# Autodesk Inventor assembly: 分析報告用
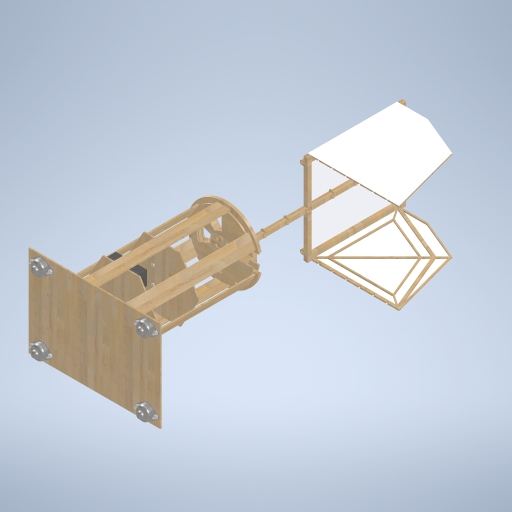
[picture p0: Inventor's stored thumbnail of the model, 512x512]
Saved by Autodesk Inventor 2024 (Build 280153000, 153)
## iProperties
Created: 2024-04-09
Part Number: 分析報告用
Document SubType Name: Assembly
Designer: USER
Author: USER
## Documents named in this file (28)
- C:\文件\機械工程實務\3D_CAD_Drawing\[Midterm]Design\分析報告用.iam
- C:\文件\機械工程實務\3D_CAD_Drawing\[Midterm]Design\cow_wheel.ipt
- C:\文件\機械工程實務\3D_CAD_Drawing\[Midterm]Design\back_down_hold.ipt
- C:\文件\機械工程實務\3D_CAD_Drawing\[Midterm]Design\back_cir_hold.ipt
- C:\文件\機械工程實務\3D_CAD_Drawing\[Midterm]Design\middle_space.ipt
- C:\文件\機械工程實務\3D_CAD_Drawing\[Midterm]Design\rolling_plate.ipt
- C:\文件\機械工程實務\3D_CAD_Drawing\[Midterm]Design\rolling_plate_top.ipt
- C:\文件\機械工程實務\3D_CAD_Drawing\[Midterm]Design\rolling_plate_small.ipt
- C:\文件\機械工程實務\3D_CAD_Drawing\[Midterm]Design\左右.ipt
- C:\文件\機械工程實務\3D_CAD_Drawing\[Midterm]Design\左右2.ipt
- C:\文件\機械工程實務\3D_CAD_Drawing\[Midterm]Design\馬達.ipt
- C:\文件\機械工程實務\3D_CAD_Drawing\[Midterm]Design\軸.ipt
- C:\文件\機械工程實務\3D_CAD_Drawing\[Midterm]Design\螺絲.ipt
- C:\文件\機械工程實務\3D_CAD_Drawing\[Midterm]Design\Base_final.ipt
- C:\文件\機械工程實務\3D_CAD_Drawing\[Midterm]Design\sail(Midterm).iam
- C:\文件\機械工程實務\3D_CAD_Drawing\[Midterm]Design\插銷B.ipt
- C:\文件\機械工程實務\3D_CAD_Drawing\[Midterm]Design\插銷A.ipt
- C:\文件\機械工程實務\3D_CAD_Drawing\[Midterm]Design\機電設備\18650電池盒\18650電池盒.ipt
- C:\文件\機械工程實務\3D_CAD_Drawing\[Midterm]Design\機電設備\馬達驅動模組\馬達驅動模組.ipt
- C:\文件\機械工程實務\3D_CAD_Drawing\[Midterm]Design\機電設備\銅柱\銅柱.ipt
- C:\文件\機械工程實務\3D_CAD_Drawing\[Midterm]Design\機電設備\Arduino板\Arduino板.iam
- C:\文件\機械工程實務\3D_CAD_Drawing\[Midterm]Design\機電設備\麵包板\麵包板.ipt
- C:\文件\機械工程實務\3D_CAD_Drawing\[Midterm]Design\機電設備\9V方型電池盒\9V方型電池盒.ipt
- C:\文件\機械工程實務\3D_CAD_Drawing\[Midterm]Design\m4螺栓.ipt
- C:\文件\機械工程實務\3D_CAD_Drawing\[Midterm]Design\middle_space2.ipt
- C:\文件\機械工程實務\3D_CAD_Drawing\[Midterm]Design\機電設備\M3螺帽\M3螺帽.ipt
- C:\文件\機械工程實務\3D_CAD_Drawing\[Midterm]Design\機電設備\M3螺栓\M3螺栓.ipt
- C:\文件\機械工程實務\3D_CAD_Drawing\[Midterm]Design\M4螺帽.ipt
## Components (70 placed, 27 different names)
1. cow_wheel:1 — 貼合:82, 貼合:83, 貼合:84, 插入:25, 插入:26
2. cow_wheel:2 — 貼合:86, 貼合:156, 貼合:157, 插入:23, 插入:24
3. cow_wheel:3 — 貼合:80, 貼合:81, 貼合:85, 插入:12, 插入:14
4. cow_wheel:4 — 貼合:75, 貼合:76, 貼合:77, 貼合:78, 貼合:79, 插入:27, 插入:28
5. back_down_hold:1 — 貼合:99, 貼合:100, 貼合:101, 貼合:102, 貼合:147
6. back_down_hold:2 — 貼合:34, 齊平:14, 相切:1, 齊平:28, 貼合:92, 貼合:93, 貼合:94
7. back_down_hold:3 — 齊平:5, 齊平:13, 貼合:90, 貼合:91, 貼合:149
8. back_down_hold:4 — 貼合:87, 貼合:97, 貼合:98
9. back_down_hold:5 — 齊平:6, 貼合:48, 貼合:88, 貼合:89, 貼合:105, 貼合:148, 齊平:44, 貼合:150, 貼合:151
10. back_down_hold:6 — 齊平:5, 齊平:6, 貼合:32, 貼合:33, 貼合:95, 貼合:96, 貼合:146, 角度:3
11. back_cir_hold:1 — 貼合:32, 貼合:33, 貼合:34, 貼合:104, 角度:1, 貼合:109
12. middle_space:1 — 齊平:13, 貼合:48, 齊平:14, 齊平:28, 貼合:145
13. rolling_plate:2 — 貼合:56, 貼合:57, 齊平:24, 貼合:104, 貼合:108, 貼合:109, 齊平:31, 貼合:135, 貼合:136, 貼合:139, 貼合:140, 貼合:141
14. rolling_plate_top:1 — 相切:1, 貼合:58, 貼合:59, 貼合:60, 貼合:61, 貼合:62, 貼合:63, 角度:1, 貼合:108, 貼合:113, 貼合:114, 貼合:115, 貼合:116, 貼合:117, 齊平:30, 貼合:118, 貼合:119, 貼合:120, 貼合:121, 貼合:122, 貼合:123, 貼合:124, 貼合:125, 貼合:126, 貼合:128, 貼合:129, 貼合:131, 貼合:132, 貼合:133, 貼合:137
15. rolling_plate_small:1 — 貼合:52, 齊平:16, 齊平:19, 貼合:56, 齊平:24
16. rolling_plate_small:2 — 貼合:52, 齊平:16, 齊平:19, 貼合:57, 貼合:107, 齊平:29
17. rolling_plate_small:4 — 貼合:107, 齊平:29, 貼合:116, 貼合:117, 齊平:30
18. 左右:1 — 貼合:58, 貼合:59, 貼合:60, 貼合:66, 貼合:67, 齊平:26, 貼合:68, 齊平:27
19. 左右2:1 — 貼合:61, 貼合:62, 貼合:63, 角度:2
20. 馬達:1 — 貼合:64, 貼合:65, 貼合:69, 貼合:70, 貼合:71
21. 軸:1 — 貼合:64, 貼合:65, 貼合:110, 貼合:111, 貼合:112
22. 螺絲:1 — 齊平:25, 貼合:66, 貼合:67, 齊平:26, 貼合:69, 貼合:70
23. 螺絲:2 — 齊平:25, 貼合:68, 齊平:27, 貼合:71
24. Base_final:1 — 貼合:75, 貼合:76, 貼合:77, 貼合:78, 貼合:79, 貼合:80, 貼合:81, 貼合:82, 貼合:83, 貼合:84, 貼合:85, 貼合:86, 貼合:87, 貼合:88, 貼合:89, 貼合:90, 貼合:91, 貼合:92, 貼合:93, 貼合:94, 貼合:95, 貼合:96, 貼合:97, 貼合:98, 貼合:99, 貼合:100, 貼合:101, 貼合:102, 貼合:105, 貼合:142, 貼合:143, 貼合:144, 齊平:40, 齊平:41, 齊平:42, 齊平:43, 插入:15, 插入:16, 插入:17, 插入:18, 插入:19, 插入:20, 插入:21, 插入:22, 貼合:156, 貼合:157
25. sail(Midterm):1 [sub-assembly] — 貼合:110, 貼合:111, 貼合:112, 角度:2
26. 插銷A:1 — 齊平:32, 貼合:127, 齊平:33, 貼合:128
27. 插銷B:2 — 貼合:123, 貼合:124, 貼合:125
28. 插銷A:2 — 貼合:138, 齊平:38, 齊平:39, 貼合:141
29. 插銷B:3 — 貼合:121, 齊平:31, 貼合:122
30. 插銷A:3 — 貼合:130, 齊平:34, 齊平:35, 貼合:131
31. 插銷B:4 — 貼合:118, 貼合:119, 貼合:120
32. 插銷A:5 — 貼合:126, 齊平:32, 貼合:127, 齊平:33, 貼合:129
33. 插銷B:6 — 貼合:113, 貼合:114, 貼合:115
34. 插銷A:6 — 貼合:134, 齊平:36, 齊平:37, 貼合:135, 貼合:136
35. 插銷A:7 — 貼合:130, 齊平:34, 齊平:35, 貼合:132, 貼合:133
36. 插銷A:8 — 貼合:138, 齊平:38, 齊平:39, 貼合:139, 貼合:140
37. 插銷A:9 — 貼合:134, 齊平:36, 齊平:37, 貼合:137
38. 18650電池盒:1 — 貼合:143, 貼合:146, 貼合:147
39. 馬達驅動模組:1 — 插入:6, 角度:3, 貼合:152, 插入:7, 貼合:154, 貼合:155
40. 銅柱:1 — 插入:2
41. Arduino板:1 [sub-assembly] — 貼合:142, 齊平:40, 齊平:41
42. 麵包板:1 — 貼合:144, 齊平:42, 齊平:43
43. 9V方型電池盒:1 — 貼合:145, 貼合:148, 貼合:149
44. middle_space2:1 — 齊平:44, 貼合:150, 貼合:151, 插入:2, 插入:3, 插入:4, 插入:5, 插入:9, 插入:10, 插入:11
45. 銅柱:2 — 插入:4, 插入:6
46. 銅柱:3 — 插入:5
47. 銅柱:4 — 插入:3, 貼合:153
48. M3螺栓:1 — 貼合:152, 貼合:153
49. M4螺帽:2 — 插入:12
50. M3螺栓:2 — 插入:7
51. M3螺栓:3 — 貼合:154
52. M3螺栓:4 — 貼合:155
53. M3螺帽:2 — 插入:9
54. M3螺帽:3 — 插入:10
55. M3螺帽:4 — 插入:11
56. M4螺帽:3 — 插入:14
57. M4螺帽:4 — 插入:23
58. M4螺帽:5 — 插入:24
59. m4螺栓:1 — 插入:15
60. m4螺栓:2 — 插入:16
61. m4螺栓:3 — 插入:19
62. m4螺栓:4 — 插入:20
63. m4螺栓:5 — 插入:17
64. m4螺栓:6 — 插入:18
65. m4螺栓:7 — 插入:22
66. m4螺栓:8 — 插入:21
67. M4螺帽:6 — 插入:25
68. M4螺帽:7 — 插入:26
69. M4螺帽:8 — 插入:27
70. M4螺帽:9 — 插入:28
## Relationships (158: Mate 102, Flush 27, Insert 25, Angle 3, Tangent 1)
- 齊平:5 [Flush]: back_down_hold:3 ↔ back_down_hold:6
- 齊平:6 [Flush]: back_down_hold:5 ↔ back_down_hold:6
- 貼合:32 [Mate]: back_down_hold:6 ↔ back_cir_hold:1
- 貼合:33 [Mate]: back_down_hold:6 ↔ back_cir_hold:1
- 貼合:34 [Mate]: back_down_hold:2 ↔ back_cir_hold:1
- 齊平:13 [Flush]: back_down_hold:3 ↔ middle_space:1
- 貼合:48 [Mate]: back_down_hold:5 ↔ middle_space:1
- 齊平:14 [Flush]: back_down_hold:2 ↔ middle_space:1
- 相切:1 [Tangent]: back_down_hold:2 ↔ rolling_plate_top:1
- 貼合:52 [Mate]: rolling_plate_small:1 ↔ rolling_plate_small:2
- 齊平:16 [Flush]: rolling_plate_small:1 ↔ rolling_plate_small:2
- 齊平:19 [Flush]: rolling_plate_small:1 ↔ rolling_plate_small:2
- 貼合:56 [Mate]: rolling_plate:2 ↔ rolling_plate_small:1
- 貼合:57 [Mate]: rolling_plate:2 ↔ rolling_plate_small:2
- 齊平:24 [Flush]: rolling_plate:2 ↔ rolling_plate_small:1
- 貼合:58 [Mate]: rolling_plate_top:1 ↔ 左右:1
- 貼合:59 [Mate]: rolling_plate_top:1 ↔ 左右:1
- 貼合:60 [Mate]: rolling_plate_top:1 ↔ 左右:1
- 貼合:61 [Mate]: rolling_plate_top:1 ↔ 左右2:1
- 貼合:62 [Mate]: rolling_plate_top:1 ↔ 左右2:1
- 貼合:63 [Mate]: rolling_plate_top:1 ↔ 左右2:1
- 貼合:64 [Mate]: 馬達:1 ↔ 軸:1
- 貼合:65 [Mate]: 馬達:1 ↔ 軸:1
- 齊平:25 [Flush]: 螺絲:1 ↔ 螺絲:2
- 貼合:66 [Mate]: 左右:1 ↔ 螺絲:1
- 貼合:67 [Mate]: 左右:1 ↔ 螺絲:1
- 齊平:26 [Flush]: 左右:1 ↔ 螺絲:1
- 貼合:68 [Mate]: 左右:1 ↔ 螺絲:2
- 齊平:27 [Flush]: 左右:1 ↔ 螺絲:2
- 貼合:69 [Mate]: 馬達:1 ↔ 螺絲:1
- 貼合:70 [Mate]: 馬達:1 ↔ 螺絲:1
- 貼合:71 [Mate]: 馬達:1 ↔ 螺絲:2
- 齊平:28 [Flush]: back_down_hold:2 ↔ middle_space:1
- 貼合:75 [Mate]: cow_wheel:4 ↔ Base_final:1
- 貼合:76 [Mate]: cow_wheel:4 ↔ Base_final:1
- 貼合:77 [Mate]: cow_wheel:4 ↔ Base_final:1
- 貼合:78 [Mate]: cow_wheel:4 ↔ Base_final:1
- 貼合:79 [Mate]: cow_wheel:4 ↔ Base_final:1
- 貼合:80 [Mate]: cow_wheel:3 ↔ Base_final:1
- 貼合:81 [Mate]: cow_wheel:3 ↔ Base_final:1
- 貼合:82 [Mate]: cow_wheel:1 ↔ Base_final:1
- 貼合:83 [Mate]: cow_wheel:1 ↔ Base_final:1
- 貼合:84 [Mate]: cow_wheel:1 ↔ Base_final:1
- 貼合:85 [Mate]: cow_wheel:3 ↔ Base_final:1
- 貼合:86 [Mate]: cow_wheel:2 ↔ Base_final:1
- 貼合:87 [Mate]: back_down_hold:4 ↔ Base_final:1
- 貼合:88 [Mate]: back_down_hold:5 ↔ Base_final:1
- 貼合:89 [Mate]: back_down_hold:5 ↔ Base_final:1
- 貼合:90 [Mate]: back_down_hold:3 ↔ Base_final:1
- 貼合:91 [Mate]: back_down_hold:3 ↔ Base_final:1
- 貼合:92 [Mate]: back_down_hold:2 ↔ Base_final:1
- 貼合:93 [Mate]: back_down_hold:2 ↔ Base_final:1
- 貼合:94 [Mate]: back_down_hold:2 ↔ Base_final:1
- 貼合:95 [Mate]: back_down_hold:6 ↔ Base_final:1
- 貼合:96 [Mate]: back_down_hold:6 ↔ Base_final:1
- 貼合:97 [Mate]: back_down_hold:4 ↔ Base_final:1
- 貼合:98 [Mate]: back_down_hold:4 ↔ Base_final:1
- 貼合:99 [Mate]: back_down_hold:1 ↔ Base_final:1
- 貼合:100 [Mate]: back_down_hold:1 ↔ Base_final:1
- 貼合:101 [Mate]: back_down_hold:1 ↔ Base_final:1
- 貼合:102 [Mate]: back_down_hold:1 ↔ Base_final:1
- 貼合:104 [Mate]: back_cir_hold:1 ↔ rolling_plate:2
- 貼合:105 [Mate]: back_down_hold:5 ↔ Base_final:1
- 角度:1 [Angle] (0 deg): back_cir_hold:1 ↔ rolling_plate_top:1
- 貼合:107 [Mate]: rolling_plate_small:2 ↔ rolling_plate_small:4
- 貼合:108 [Mate]: rolling_plate:2 ↔ rolling_plate_top:1
- 齊平:29 [Flush]: rolling_plate_small:2 ↔ rolling_plate_small:4
- 貼合:109 [Mate] (1.5 mm): back_cir_hold:1 ↔ rolling_plate:2
- 貼合:110 [Mate]: 軸:1 ↔ sail(Midterm):1
- 貼合:111 [Mate]: 軸:1 ↔ sail(Midterm):1
- 貼合:112 [Mate]: 軸:1 ↔ sail(Midterm):1
- 貼合:113 [Mate]: rolling_plate_top:1 ↔ 插銷B:6
- 貼合:114 [Mate]: rolling_plate_top:1 ↔ 插銷B:6
- 貼合:115 [Mate]: rolling_plate_top:1 ↔ 插銷B:6
- 貼合:116 [Mate]: rolling_plate_top:1 ↔ rolling_plate_small:4
- 貼合:117 [Mate]: rolling_plate_top:1 ↔ rolling_plate_small:4
- 齊平:30 [Flush]: rolling_plate_top:1 ↔ rolling_plate_small:4
- 貼合:118 [Mate]: rolling_plate_top:1 ↔ 插銷B:4
- 貼合:119 [Mate]: rolling_plate_top:1 ↔ 插銷B:4
- 貼合:120 [Mate]: rolling_plate_top:1 ↔ 插銷B:4
- 貼合:121 [Mate]: rolling_plate_top:1 ↔ 插銷B:3
- 齊平:31 [Flush]: rolling_plate:2 ↔ 插銷B:3
- 貼合:122 [Mate]: rolling_plate_top:1 ↔ 插銷B:3
- 貼合:123 [Mate]: rolling_plate_top:1 ↔ 插銷B:2
- 貼合:124 [Mate]: rolling_plate_top:1 ↔ 插銷B:2
- 貼合:125 [Mate]: rolling_plate_top:1 ↔ 插銷B:2
- 貼合:126 [Mate]: rolling_plate_top:1 ↔ 插銷A:5
- 齊平:32 [Flush]: 插銷A:1 ↔ 插銷A:5
- 貼合:127 [Mate]: 插銷A:1 ↔ 插銷A:5
- 齊平:33 [Flush]: 插銷A:1 ↔ 插銷A:5
- 貼合:128 [Mate]: rolling_plate_top:1 ↔ 插銷A:1
- 貼合:129 [Mate]: rolling_plate_top:1 ↔ 插銷A:5
- 貼合:130 [Mate]: 插銷A:3 ↔ 插銷A:7
- 齊平:34 [Flush]: 插銷A:3 ↔ 插銷A:7
- 齊平:35 [Flush]: 插銷A:3 ↔ 插銷A:7
- 貼合:131 [Mate]: rolling_plate_top:1 ↔ 插銷A:3
- 貼合:132 [Mate]: rolling_plate_top:1 ↔ 插銷A:7
- 貼合:133 [Mate]: rolling_plate_top:1 ↔ 插銷A:7
- 貼合:134 [Mate]: 插銷A:6 ↔ 插銷A:9
- 齊平:36 [Flush]: 插銷A:6 ↔ 插銷A:9
- 齊平:37 [Flush]: 插銷A:6 ↔ 插銷A:9
- 貼合:135 [Mate]: rolling_plate:2 ↔ 插銷A:6
- 貼合:136 [Mate]: rolling_plate:2 ↔ 插銷A:6
- 貼合:137 [Mate]: rolling_plate_top:1 ↔ 插銷A:9
- 貼合:138 [Mate]: 插銷A:2 ↔ 插銷A:8
- 齊平:38 [Flush]: 插銷A:2 ↔ 插銷A:8
- 齊平:39 [Flush]: 插銷A:2 ↔ 插銷A:8
- 貼合:139 [Mate]: rolling_plate:2 ↔ 插銷A:8
- 貼合:140 [Mate]: rolling_plate:2 ↔ 插銷A:8
- 貼合:141 [Mate]: rolling_plate:2 ↔ 插銷A:2
- 角度:2 [Angle] (0 deg): 左右2:1 ↔ sail(Midterm):1
- 貼合:142 [Mate]: Base_final:1 ↔ Arduino板:1
- 貼合:143 [Mate]: Base_final:1 ↔ 18650電池盒:1
- 貼合:144 [Mate]: Base_final:1 ↔ 麵包板:1
- 貼合:145 [Mate]: middle_space:1 ↔ 9V方型電池盒:1
- 齊平:40 [Flush] (40 mm): Base_final:1 ↔ Arduino板:1
- 齊平:41 [Flush] (30 mm): Base_final:1 ↔ Arduino板:1
- 齊平:42 [Flush] (55 mm): Base_final:1 ↔ 麵包板:1
- 齊平:43 [Flush] (25 mm): Base_final:1 ↔ 麵包板:1
- 貼合:146 [Mate] (30.7 mm): back_down_hold:6 ↔ 18650電池盒:1
- 貼合:147 [Mate] (27.422 mm): back_down_hold:1 ↔ 18650電池盒:1
- 貼合:148 [Mate]: back_down_hold:5 ↔ 9V方型電池盒:1
- 貼合:149 [Mate] (19.072 mm): back_down_hold:3 ↔ 9V方型電池盒:1
- 齊平:44 [Flush]: back_down_hold:5 ↔ middle_space2:1
- 貼合:150 [Mate]: back_down_hold:5 ↔ middle_space2:1
- 貼合:151 [Mate]: back_down_hold:5 ↔ middle_space2:1
- 插入:2 [Insert]: 銅柱:1 ↔ middle_space2:1
- 插入:3 [Insert]: middle_space2:1 ↔ 銅柱:4
- 插入:4 [Insert]: middle_space2:1 ↔ 銅柱:2
- 插入:5 [Insert]: middle_space2:1 ↔ 銅柱:3
- 插入:6 [Insert]: 馬達驅動模組:1 ↔ 銅柱:2
- 角度:3 [Angle] (180 deg): back_down_hold:6 ↔ 馬達驅動模組:1
- 貼合:152 [Mate]: 馬達驅動模組:1 ↔ M3螺栓:1
- 貼合:153 [Mate]: 銅柱:4 ↔ M3螺栓:1
- 插入:7 [Insert]: 馬達驅動模組:1 ↔ M3螺栓:2
- 貼合:154 [Mate]: 馬達驅動模組:1 ↔ M3螺栓:3
- 貼合:155 [Mate]: 馬達驅動模組:1 ↔ M3螺栓:4
- 插入:9 [Insert]: middle_space2:1 ↔ M3螺帽:2
- 插入:10 [Insert]: middle_space2:1 ↔ M3螺帽:3
- 插入:11 [Insert]: middle_space2:1 ↔ M3螺帽:4
- 插入:12 [Insert]: cow_wheel:3 ↔ M4螺帽:2
- 插入:14 [Insert]: cow_wheel:3 ↔ M4螺帽:3
- 插入:15 [Insert]: Base_final:1 ↔ m4螺栓:1
- 插入:16 [Insert]: Base_final:1 ↔ m4螺栓:2
- 插入:17 [Insert]: Base_final:1 ↔ m4螺栓:5
- 插入:18 [Insert]: Base_final:1 ↔ m4螺栓:6
- 插入:19 [Insert]: Base_final:1 ↔ m4螺栓:3
- 插入:20 [Insert]: Base_final:1 ↔ m4螺栓:4
- 插入:21 [Insert]: Base_final:1 ↔ m4螺栓:8
- 插入:22 [Insert]: Base_final:1 ↔ m4螺栓:7
- 貼合:156 [Mate]: cow_wheel:2 ↔ Base_final:1
- 貼合:157 [Mate]: cow_wheel:2 ↔ Base_final:1
- 插入:23 [Insert]: cow_wheel:2 ↔ M4螺帽:4
- 插入:24 [Insert]: cow_wheel:2 ↔ M4螺帽:5
- 插入:25 [Insert]: cow_wheel:1 ↔ M4螺帽:6
- 插入:26 [Insert]: cow_wheel:1 ↔ M4螺帽:7
- 插入:27 [Insert]: cow_wheel:4 ↔ M4螺帽:8
- 插入:28 [Insert]: cow_wheel:4 ↔ M4螺帽:9
